# Autodesk Inventor assembly: Base2
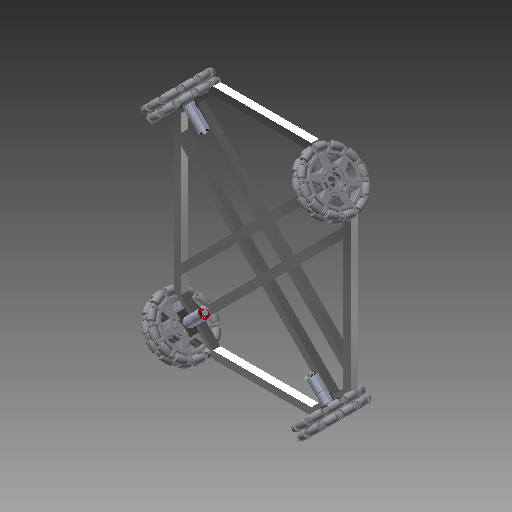
[picture p0: Inventor's stored thumbnail of the model, 512x512]
Saved by Autodesk Inventor 2017 SP1 (Build 210196100, 196)
## iProperties
Created: 2017-06-13
Part Number: Base2
Document SubType Name: Assembly
Designer: zallen
Author: zallen
## Documents named in this file (3)
- C:\Users\Zach\Documents\GitHub\cr-laundry-robot\src\Base 2\Base2.iam
- C:\Users\Zach\Documents\GitHub\cr-laundry-robot\src\Base 2\Chassis\Chassis.iam
- C:\Users\Zach\Documents\GitHub\cr-laundry-robot\lib\DC Motor with Encoder\Motor.ipt
## Components (5 placed, 2 different names)
1. Chassis:1 [sub-assembly] — Mate:1, Mate:2, Mate:3, Mate:4, Mate:5, Mate:6, Mate:7, Mate:8
2. Motor:1 — Mate:1, Mate:2
3. Motor:2 — Mate:7, Mate:8
4. Motor:3 — Mate:5, Mate:6
5. Motor:4 — Mate:3, Mate:4
## Relationships (8: Mate 8)
- Mate:1: Chassis:1 ↔ Motor:1
- Mate:2: Chassis:1 ↔ Motor:1
- Mate:3: Chassis:1 ↔ Motor:4
- Mate:4: Chassis:1 ↔ Motor:4
- Mate:5: Chassis:1 ↔ Motor:3
- Mate:6: Chassis:1 ↔ Motor:3
- Mate:7: Chassis:1 ↔ Motor:2
- Mate:8: Chassis:1 ↔ Motor:2
